# Autodesk Inventor assembly: Etau
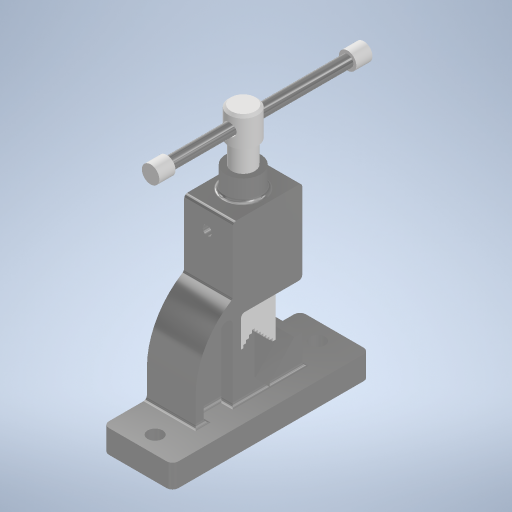
[picture p0: Inventor's stored thumbnail of the model, 512x512]
Saved by Autodesk Inventor 2023.2 (Build 272271030, 271C)
## iProperties
Created: 2023-03-08
Part Number: Etau
Document SubType Name: Assembly
Designer: Luis Valente
Author: Luis Valente
## Documents named in this file (6)
- C:\Users\lc010\OneDrive\Documentos\Henallux\Inventor School\Etau pour tubes\Etau.iam
- C:\Users\lc010\OneDrive\Documentos\Henallux\Inventor School\Etau pour tubes\Corps\Corps.ipt
- C:\Users\lc010\OneDrive\Documentos\Henallux\Inventor School\Etau pour tubes\Machoire\Machoire.ipt
- C:\Users\lc010\OneDrive\Documentos\Henallux\Inventor School\Etau pour tubes\Vis\Vis de manoeuvre.ipt
- C:\Users\lc010\OneDrive\Documentos\Henallux\Inventor School\Etau pour tubes\Manivelle et embouts\Manivelle.ipt
- C:\Users\lc010\OneDrive\Documentos\Henallux\Inventor School\Etau pour tubes\Manivelle et embouts\Embouts.ipt
## Components (6 placed, 5 different names)
1. Corps:1 — Cylindrical:1
2. Vis de manoeuvre:1 — Cylindrical:1, Rigid:5, Cylindrical:7
3. Machoire:1 — Rigid:5
4. Manivelle:1 — Cylindrical:5, Cylindrical:6, Mate:1, Mate:2, Cylindrical:7
5. Embouts:1 — Cylindrical:5, Mate:1
6. Embouts:2 — Cylindrical:6, Mate:2
## Relationships (7: CylindricalJoint 4, Mate 2, WeldJoint 1)
- Cylindrical:1: Corps:1 ↔ Vis de manoeuvre:1
- Cylindrical:5: Manivelle:1 ↔ Embouts:1
- Cylindrical:6: Manivelle:1 ↔ Embouts:2
- Rigid:5 [WeldJoint] (-20 mm): Vis de manoeuvre:1 ↔ Machoire:1
- Mate:1: Manivelle:1 ↔ Embouts:1
- Mate:2: Manivelle:1 ↔ Embouts:2
- Cylindrical:7: Vis de manoeuvre:1 ↔ Manivelle:1
